# Autodesk Inventor assembly: OpenHFNC-1
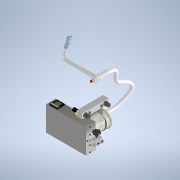
[picture p0: Inventor's stored thumbnail of the model, 180x180]
Saved by Autodesk Inventor 2020.3 (Build 243373000, 373)
## iProperties
Created: 2020-08-07
Part Number: OpenHFNC-1
Document SubType Name: Assembly
Designer: Bruno
Author: Bruno
## Documents named in this file (45)
- C:\Users\Bruno\Desktop\CAD GH3\Inventor\OpenHFNC-1.iam
- C:\Users\Bruno\Desktop\CAD GH3\Inventor\Heating Box\Heating plate box\Box base.ipt
- C:\Users\Bruno\Desktop\CAD GH3\Inventor\Heating Box\Heating plate box\M4 Rivet nut.ipt
- C:\Users\Bruno\Desktop\CAD GH3\Inventor\Heating Box\Heating plate box\Box top.ipt
- C:\Users\Bruno\Desktop\CAD GH3\Inventor\Heating Box\Heating plate box\DIN912 M4x0.7x10-8.8 socket head screw.ipt
- C:\Users\Bruno\Desktop\CAD GH3\Inventor\Heating Box\Heating plate box\Oring 2-343 Silicone.ipt
- C:\Users\Bruno\Desktop\CAD GH3\Inventor\Heating Box\Heating plate box\Heating plate.ipt
- C:\Users\Bruno\Desktop\CAD GH3\Inventor\Heating Box\Heating plate box\Heater Fixing Bar.ipt
- C:\Users\Bruno\Desktop\CAD GH3\Inventor\Heating Box\Heating plate box\DIN912 M4x0.7x40-8.8 socket head screw.ipt
- C:\Users\Bruno\Desktop\CAD GH3\Inventor\Heating Box\Heating plate box\DIN934-M4 nut.ipt
- C:\Users\Bruno\Desktop\CAD GH3\Inventor\Heating Box\Electric parts\Heater630W.ipt
- C:\Users\Bruno\Desktop\CAD GH3\Inventor\Heating Box\Electric parts\Thermocouple.ipt
- C:\Users\Bruno\Desktop\CAD GH3\Inventor\Heating Box\Electric parts\RexC100 controller.ipt
- C:\Users\Bruno\Desktop\CAD GH3\Inventor\Heating Box\Electric parts\IEC C14 Male panel connector.ipt
- C:\Users\Bruno\Desktop\CAD GH3\Inventor\Heating Box\Electric parts\DIN7991 M3x0.5x10-8.8 countersunk head cap screws.ipt
- C:\Users\Bruno\Desktop\CAD GH3\Inventor\Heating Box\Electric parts\DIN934-M3 nut.ipt
- C:\Users\Bruno\Desktop\CAD GH3\Inventor\Heating Box\Electric parts\On-Off Switch.ipt
- C:\Users\Bruno\Desktop\CAD GH3\Inventor\Heating Box\Electric parts\Solid State Relay SSR40DA.ipt
- C:\Users\Bruno\Desktop\CAD GH3\Inventor\Heating Box\Electric parts\220 AC power cable.ipt
- C:\Users\Bruno\Desktop\CAD GH3\Inventor\Heating Box\Glass vase _ flow meter fixer\Glass fixer plate.ipt
- C:\Users\Bruno\Desktop\CAD GH3\Inventor\Heating Box\Glass vase _ flow meter fixer\DIN912 M4x0.7x10-8.8 socket head screw.ipt
- C:\Users\Bruno\Desktop\CAD GH3\Inventor\Heating Box\Glass vase _ flow meter fixer\Oring 2-159 for glassfixer.ipt
- C:\Users\Bruno\Desktop\CAD GH3\Inventor\Heating Box\IV stand fixer\IV stand fixer plate.ipt
- C:\Users\Bruno\Desktop\CAD GH3\Inventor\Heating Box\IV stand fixer\DIN912 M4x0.7x10-8.8 socket head screw.ipt
- C:\Users\Bruno\Desktop\CAD GH3\Inventor\Heating Box\IV stand fixer\Split Washer DIN127B D4.ipt
- C:\Users\Bruno\Desktop\CAD GH3\Inventor\Heating Box\IV stand fixer\DIN934-M4 nut.ipt
- C:\Users\Bruno\Desktop\CAD GH3\Inventor\Heating Box\IV stand fixer\Star Knob 1-4UNC.ipt
- C:\Users\Bruno\Desktop\CAD GH3\Inventor\Ventilation pipeline\Flow pipelines\LZM-15ZT flowmeter.iam
- C:\Users\Bruno\Desktop\CAD GH3\Inventor\Ventilation pipeline\Beaker glass - top connector\Beaker glass 600ml, diam_ 90mm.ipt
- C:\Users\Bruno\Desktop\CAD GH3\Inventor\Ventilation pipeline\Beaker glass - top connector\Top lid body.ipt
- C:\Users\Bruno\Desktop\CAD GH3\Inventor\Ventilation pipeline\Beaker glass - top connector\Paddle.ipt
- C:\Users\Bruno\Desktop\CAD GH3\Inventor\Ventilation pipeline\Beaker glass - top connector\Oring 2-007.ipt
- C:\Users\Bruno\Desktop\CAD GH3\Inventor\Ventilation pipeline\Beaker glass - top connector\DIN912 M4x0.7x16-8.8 socket head screw.ipt
- C:\Users\Bruno\Desktop\CAD GH3\Inventor\Ventilation pipeline\Beaker glass - top connector\Oring 2-026.ipt
- C:\Users\Bruno\Desktop\CAD GH3\Inventor\Ventilation pipeline\Beaker glass - top connector\Oring 2-019.ipt
- C:\Users\Bruno\Desktop\CAD GH3\Inventor\Ventilation pipeline\Beaker glass - top connector\Oring 2-151_D.ipt
- C:\Users\Bruno\Desktop\CAD GH3\Inventor\Ventilation pipeline\Beaker glass - top connector\Corrugated tube-top lid connector.ipt
- C:\Users\Bruno\Desktop\CAD GH3\Inventor\Ventilation pipeline\Beaker glass - top connector\Heated tube-top lid connector.ipt
- C:\Users\Bruno\Desktop\CAD GH3\Inventor\Ventilation pipeline\Beaker glass - top connector\Oring 2-018_D.ipt
- C:\Users\Bruno\Desktop\CAD GH3\Inventor\Ventilation pipeline\Beaker glass - top connector\Oring 2-022.ipt
- C:\Users\Bruno\Desktop\CAD GH3\Inventor\Ventilation pipeline\Flow pipelines\Heated Tube (short version).ipt
- C:\Users\Bruno\Desktop\CAD GH3\Inventor\Ventilation pipeline\Flow pipelines\Transfer tube (bended version).ipt
- C:\Users\Bruno\Desktop\CAD GH3\Inventor\Ventilation pipeline\Flow pipelines\Conical rubber stopper.ipt
- C:\Users\Bruno\Desktop\CAD GH3\Inventor\Ventilation pipeline\Nasal cannula\Nasal Cannula.ipt
- C:\Users\Bruno\Desktop\CAD GH3\Inventor\Ventilation pipeline\Nasal cannula\Oring 2-014.ipt
## Components (81 placed, 41 different names)
1. Box base:1 — Insert:1, Insert:2, Insert:3, Insert:4, Insert:5, Insert:6, Insert:7, Insert:8, Insert:9, Insert:10, Insert:11, Insert:12, Cylindrical:8, Cylindrical:9, Cylindrical:12, Cylindrical:13, Cylindrical:14, Mate:3, Mate:4, Mate:5
2. M4 Rivet nut:1 — Insert:6
3. M4 Rivet nut:2 — Insert:7
4. M4 Rivet nut:3 — Insert:4
5. M4 Rivet nut:4 — Insert:5, Mate:1
6. M4 Rivet nut:5 — Insert:3
7. M4 Rivet nut:6 — Insert:2
8. M4 Rivet nut:7 — Insert:1
9. M4 Rivet nut:8 — Insert:12
10. M4 Rivet nut:9 — Insert:11
11. M4 Rivet nut:10 — Insert:10, Insert:13
12. M4 Rivet nut:11 — Insert:8, Cylindrical:15
13. M4 Rivet nut:12 — Insert:9
14. Box top:1 — Mate:1, Insert:13, Insert:14, Insert:15, Insert:16, Insert:17, Insert:19, Insert:20, Insert:21, Insert:22, Insert:23, Insert:24, Insert:25, Insert:26, Insert:27, Insert:28, Cylindrical:1, Cylindrical:3, Insert:29, Insert:30
15. M4 Rivet nut:13 — Insert:16
16. M4 Rivet nut:14 — Insert:17
17. M4 Rivet nut:15 — Insert:14, Cylindrical:17
18. M4 Rivet nut:16 — Insert:15, Cylindrical:18
19. DIN912 M4x0.7x10-8.8 socket head screw:1 — Insert:20
20. DIN912 M4x0.7x10-8.8 socket head screw:2 — Insert:19
21. DIN912 M4x0.7x10-8.8 socket head screw:3 — Insert:21
22. DIN912 M4x0.7x10-8.8 socket head screw:4 — Insert:26
23. DIN912 M4x0.7x10-8.8 socket head screw:5 — Insert:27
24. DIN912 M4x0.7x10-8.8 socket head screw:6 — Insert:28
25. DIN912 M4x0.7x10-8.8 socket head screw:7 — Insert:24
26. DIN912 M4x0.7x10-8.8 socket head screw:8 — Insert:25
27. DIN912 M4x0.7x10-8.8 socket head screw:9 — Insert:23
28. DIN912 M4x0.7x10-8.8 socket head screw:10 — Insert:22
29. Oring 2-343 Silicone:1 — Cylindrical:1, Cylindrical:2
30. Heating plate:1 — Cylindrical:2, Mate:2, Cylindrical:6, Cylindrical:7, Cylindrical:21
31. Heater Fixing Bar:1 — Mate:2, Cylindrical:3, Cylindrical:4, Cylindrical:5
32. DIN912 M4x0.7x40-8.8 socket head screw:1 — Insert:29
33. DIN912 M4x0.7x40-8.8 socket head screw:2 — Insert:30
34. DIN934-M4 nut:1 — Cylindrical:4
35. DIN934-M4 nut:2 — Cylindrical:5
36. Heater630W:1 — Cylindrical:6
37. Thermocouple:1 — Cylindrical:7
38. RexC100 controller:1 — Cylindrical:8
39. IEC C14 Male panel connector:1 — Cylindrical:9, Cylindrical:10, Cylindrical:11, Mate:6, Mate:7, Mate:8
40. DIN7991 M3x0.5x10-8.8 countersunk head cap screws:1 — Cylindrical:11
41. DIN7991 M3x0.5x10-8.8 countersunk head cap screws:2 — Cylindrical:10
42. DIN934-M3 nut:1 — Cylindrical:12
43. DIN934-M3 nut:2 — Cylindrical:13
44. On-Off Switch:1 — Cylindrical:14
45. SSR-XXDA:1 — Mate:3, Mate:4, Mate:5
46. 220 AC power cable:1 — Mate:6, Mate:7, Mate:8
47. Glass fixer plate:1 — Cylindrical:15, Insert:31, Insert:32, Cylindrical:16, Cylindrical:20, Angle:1
48. DIN912 M4x0.7x10-8.8 socket head screw:11 — Insert:31
49. DIN912 M4x0.7x10-8.8 socket head screw:12 — Insert:32
50. Oring 2-159 for glassfixer:1 — Cylindrical:16
51. IV stand fixer plate:1 — Cylindrical:17, Insert:33, Insert:34, Insert:37, Insert:38, Cylindrical:19
52. IV stand fixer plate:2 — Cylindrical:18, Insert:35, Insert:36, Insert:41, Insert:42
53. DIN912 M4x0.7x10-8.8 socket head screw:13 — Insert:39
54. DIN912 M4x0.7x10-8.8 socket head screw:14 — Insert:40
55. DIN912 M4x0.7x10-8.8 socket head screw:15 — Insert:36
56. DIN912 M4x0.7x10-8.8 socket head screw:16 — Insert:35
57. DIN912 M4x0.7x10-8.8 socket head screw:17 — Insert:34
58. DIN912 M4x0.7x10-8.8 socket head screw:18 — Insert:33
59. Split Washer DIN127B D4:1 — Insert:38, Insert:39
60. Split Washer DIN127B D4:2 — Insert:37, Insert:40
61. DIN934-M4 nut:3 — Insert:41
62. DIN934-M4 nut:4 — Insert:42
63. Star Knob 1-4UNC:1 — Cylindrical:19
64. LZM-15ZT flowmeter:1 [sub-assembly] — Cylindrical:20, Angle:1
65. Beaker glass 600ml, diam_ 90mm:1 — Cylindrical:21, Cylindrical:31
66. Top lid body:1 — Cylindrical:22, Cylindrical:23, Rigid:1, Cylindrical:25, Cylindrical:26, Cylindrical:27, Cylindrical:28, Cylindrical:31
67. Paddle:1 — Cylindrical:22
68. Oring 2-007:1 — Cylindrical:23, Cylindrical:24
69. DIN912 M4x0.7x16-8.8 socket head screw:1 — Cylindrical:24
70. Oring 2-026:1 — Rigid:1
71. Oring 2-019:1 — Cylindrical:25
72. Oring 2-151_D:1 — Cylindrical:26
73. Corrugated tube-top lid connector:1 — Cylindrical:27, Cylindrical:30
74. Heated tube-top lid connector:1 — Cylindrical:28, Cylindrical:29, Cylindrical:32
75. Oring 2-018_D:1 — Cylindrical:30
76. Oring 2-022:1 — Cylindrical:29
77. Heated Tube (short version):1 — Cylindrical:32, Cylindrical:33
78. Transfer tube (bended version):1 — Cylindrical:33, Cylindrical:34, Cylindrical:36
79. Conical rubber stopper:1 — Cylindrical:34
80. Nasal Cannula:1 — Cylindrical:35, Cylindrical:36
81. Oring 2-014:1 — Cylindrical:35
## Relationships (87: Insert 41, CylindricalJoint 36, Mate 8, Angle 1, WeldJoint 1)
- Insert:1: Box base:1 ↔ M4 Rivet nut:7
- Insert:2: Box base:1 ↔ M4 Rivet nut:6
- Insert:3: Box base:1 ↔ M4 Rivet nut:5
- Insert:4: Box base:1 ↔ M4 Rivet nut:3
- Insert:5: Box base:1 ↔ M4 Rivet nut:4
- Insert:6: Box base:1 ↔ M4 Rivet nut:1
- Insert:7: Box base:1 ↔ M4 Rivet nut:2
- Insert:8: Box base:1 ↔ M4 Rivet nut:11
- Insert:9: Box base:1 ↔ M4 Rivet nut:12
- Insert:10: Box base:1 ↔ M4 Rivet nut:10
- Insert:11: Box base:1 ↔ M4 Rivet nut:9
- Insert:12: Box base:1 ↔ M4 Rivet nut:8
- Mate:1: M4 Rivet nut:4 ↔ Box top:1
- Insert:13: M4 Rivet nut:10 ↔ Box top:1
- Insert:14: Box top:1 ↔ M4 Rivet nut:15
- Insert:15: Box top:1 ↔ M4 Rivet nut:16
- Insert:16: Box top:1 ↔ M4 Rivet nut:13
- Insert:17: Box top:1 ↔ M4 Rivet nut:14
- Insert:19: Box top:1 ↔ DIN912 M4x0.7x10-8.8 socket head screw:2
- Insert:20: Box top:1 ↔ DIN912 M4x0.7x10-8.8 socket head screw:1
- Insert:21: Box top:1 ↔ DIN912 M4x0.7x10-8.8 socket head screw:3
- Insert:22: Box top:1 ↔ DIN912 M4x0.7x10-8.8 socket head screw:10
- Insert:23: Box top:1 ↔ DIN912 M4x0.7x10-8.8 socket head screw:9
- Insert:24: Box top:1 ↔ DIN912 M4x0.7x10-8.8 socket head screw:7
- Insert:25: Box top:1 ↔ DIN912 M4x0.7x10-8.8 socket head screw:8
- Insert:26: Box top:1 ↔ DIN912 M4x0.7x10-8.8 socket head screw:4
- Insert:27: Box top:1 ↔ DIN912 M4x0.7x10-8.8 socket head screw:5
- Insert:28: Box top:1 ↔ DIN912 M4x0.7x10-8.8 socket head screw:6
- Cylindrical:1: Box top:1 ↔ Oring 2-343 Silicone:1
- Cylindrical:2: Oring 2-343 Silicone:1 ↔ Heating plate:1
- Mate:2: Heating plate:1 ↔ Heater Fixing Bar:1
- Cylindrical:3: Box top:1 ↔ Heater Fixing Bar:1
- Insert:29: Box top:1 ↔ DIN912 M4x0.7x40-8.8 socket head screw:1
- Insert:30: Box top:1 ↔ DIN912 M4x0.7x40-8.8 socket head screw:2
- Cylindrical:4: Heater Fixing Bar:1 ↔ DIN934-M4 nut:1
- Cylindrical:5: Heater Fixing Bar:1 ↔ DIN934-M4 nut:2
- Cylindrical:6: Heating plate:1 ↔ Heater630W:1
- Cylindrical:7: Heating plate:1 ↔ Thermocouple:1
- Cylindrical:8: Box base:1 ↔ RexC100 controller:1
- Cylindrical:9: Box base:1 ↔ IEC C14 Male panel connector:1
- Cylindrical:10: IEC C14 Male panel connector:1 ↔ DIN7991 M3x0.5x10-8.8 countersunk head cap screws:2
- Cylindrical:11: IEC C14 Male panel connector:1 ↔ DIN7991 M3x0.5x10-8.8 countersunk head cap screws:1
- Cylindrical:12: Box base:1 ↔ DIN934-M3 nut:1
- Cylindrical:13: Box base:1 ↔ DIN934-M3 nut:2
- Cylindrical:14: Box base:1 ↔ On-Off Switch:1
- Mate:3: Box base:1 ↔ SSR-XXDA:1
- Mate:4 (10 mm): Box base:1 ↔ SSR-XXDA:1
- Mate:5 (5 mm): Box base:1 ↔ SSR-XXDA:1
- Mate:6: IEC C14 Male panel connector:1 ↔ 220 AC power cable:1
- Mate:7: IEC C14 Male panel connector:1 ↔ 220 AC power cable:1
- Mate:8: IEC C14 Male panel connector:1 ↔ 220 AC power cable:1
- Cylindrical:15: M4 Rivet nut:11 ↔ Glass fixer plate:1
- Insert:31: Glass fixer plate:1 ↔ DIN912 M4x0.7x10-8.8 socket head screw:11
- Insert:32: Glass fixer plate:1 ↔ DIN912 M4x0.7x10-8.8 socket head screw:12
- Cylindrical:16: Glass fixer plate:1 ↔ Oring 2-159 for glassfixer:1
- Cylindrical:17: M4 Rivet nut:15 ↔ IV stand fixer plate:1
- Cylindrical:18: M4 Rivet nut:16 ↔ IV stand fixer plate:2
- Insert:33: IV stand fixer plate:1 ↔ DIN912 M4x0.7x10-8.8 socket head screw:18
- Insert:34: IV stand fixer plate:1 ↔ DIN912 M4x0.7x10-8.8 socket head screw:17
- Insert:35: IV stand fixer plate:2 ↔ DIN912 M4x0.7x10-8.8 socket head screw:16
- Insert:36: IV stand fixer plate:2 ↔ DIN912 M4x0.7x10-8.8 socket head screw:15
- Insert:37: IV stand fixer plate:1 ↔ Split Washer DIN127B D4:2
- Insert:38: IV stand fixer plate:1 ↔ Split Washer DIN127B D4:1
- Insert:39: DIN912 M4x0.7x10-8.8 socket head screw:13 ↔ Split Washer DIN127B D4:1
- Insert:40: DIN912 M4x0.7x10-8.8 socket head screw:14 ↔ Split Washer DIN127B D4:2
- Insert:41: IV stand fixer plate:2 ↔ DIN934-M4 nut:3
- Insert:42: IV stand fixer plate:2 ↔ DIN934-M4 nut:4
- Cylindrical:19: IV stand fixer plate:1 ↔ Star Knob 1-4UNC:1
- Cylindrical:20: Glass fixer plate:1 ↔ LZM-15ZT flowmeter:1
- Angle:1 (0 deg): Glass fixer plate:1 ↔ LZM-15ZT flowmeter:1
- Cylindrical:21: Heating plate:1 ↔ Beaker glass 600ml, diam_ 90mm:1
- Cylindrical:22: Top lid body:1 ↔ Paddle:1
- Cylindrical:23: Top lid body:1 ↔ Oring 2-007:1
- Cylindrical:24: Oring 2-007:1 ↔ DIN912 M4x0.7x16-8.8 socket head screw:1
- Rigid:1 [WeldJoint] (-1.5 mm): Top lid body:1 ↔ Oring 2-026:1
- Cylindrical:25: Top lid body:1 ↔ Oring 2-019:1
- Cylindrical:26: Top lid body:1 ↔ Oring 2-151_D:1
- Cylindrical:27: Top lid body:1 ↔ Corrugated tube-top lid connector:1
- Cylindrical:28: Top lid body:1 ↔ Heated tube-top lid connector:1
- Cylindrical:29: Heated tube-top lid connector:1 ↔ Oring 2-022:1
- Cylindrical:30: Corrugated tube-top lid connector:1 ↔ Oring 2-018_D:1
- Cylindrical:31: Beaker glass 600ml, diam_ 90mm:1 ↔ Top lid body:1
- Cylindrical:32: Heated tube-top lid connector:1 ↔ Heated Tube (short version):1
- Cylindrical:33: Heated Tube (short version):1 ↔ Transfer tube (bended version):1
- Cylindrical:34: Transfer tube (bended version):1 ↔ Conical rubber stopper:1
- Cylindrical:35: Nasal Cannula:1 ↔ Oring 2-014:1
- Cylindrical:36: Transfer tube (bended version):1 ↔ Nasal Cannula:1
